# Autodesk Inventor assembly: actuator assembly
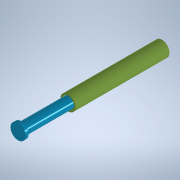
[picture p0: Inventor's stored thumbnail of the model, 180x180]
Saved by Autodesk Inventor 2020 (Build 240168000, 168)
## iProperties
Created: 2020-12-11
Part Number: actuator assembly
Document SubType Name: Assembly
Designer: Vikki
Author: Vikki
## Documents named in this file (3)
- E:\borewell rescuebot\pll manipulator files\sps manipulator\actuator assembly.iam
- E:\borewell rescuebot\pll manipulator files\sps manipulator\piston v1.ipt
- E:\borewell rescuebot\pll manipulator files\sps manipulator\plunger v1.ipt
## Components (2 placed, 2 different names)
1. piston v1:2 — Mate:1
2. plunger v1:1 — Mate:1
## Relationships (1: Mate 1)
- Mate:1: piston v1:2 ↔ plunger v1:1
